# Autodesk Inventor assembly: multipurpose_distiller_assembly
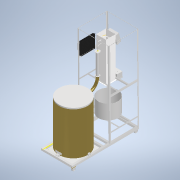
[picture p0: Inventor's stored thumbnail of the model, 180x180]
Saved by Autodesk Inventor 2020 (Build 240168000, 168)
## iProperties
Created: 2022-09-01
Part Number: multipurpose_distiller_assembly
Document SubType Name: Assembly
Designer: Intuito_PC
Author: Intuito_PC
## Documents named in this file (18)
- C:\Users\Intuito_PC\Desktop\academ\final_yr_project\auto_distiller\report_work\Project_Implementation_Report\CAD\multipurpose_distiller_assembly.iam
- C:\Users\Intuito_PC\Desktop\academ\final_yr_project\auto_distiller\report_work\Project_Implementation_Report\CAD\frame.ipt
- C:\Users\Intuito_PC\Desktop\academ\final_yr_project\auto_distiller\report_work\Project_Implementation_Report\CAD\still.ipt
- C:\Users\Intuito_PC\Desktop\academ\final_yr_project\auto_distiller\report_work\Project_Implementation_Report\CAD\fractionating_column.ipt
- C:\Users\Intuito_PC\Desktop\academ\final_yr_project\auto_distiller\report_work\Project_Implementation_Report\CAD\fractionating_column_cover.ipt
- C:\Users\Intuito_PC\Desktop\academ\final_yr_project\auto_distiller\report_work\Project_Implementation_Report\CAD\condenser.ipt
- C:\Users\Intuito_PC\Desktop\academ\final_yr_project\auto_distiller\report_work\Project_Implementation_Report\CAD\AC_heater_coil.ipt
- C:\Users\Intuito_PC\Desktop\academ\final_yr_project\auto_distiller\report_work\Project_Implementation_Report\CAD\AC_power_box.ipt
- C:\Users\Intuito_PC\Desktop\academ\final_yr_project\auto_distiller\report_work\Project_Implementation_Report\CAD\boiler_plates.ipt
- C:\Users\Intuito_PC\Desktop\academ\final_yr_project\auto_distiller\report_work\Project_Implementation_Report\CAD\control_panel_box.ipt
- C:\Users\Intuito_PC\Desktop\academ\final_yr_project\auto_distiller\report_work\Project_Implementation_Report\CAD\oil_water_separator.ipt
- C:\Users\Intuito_PC\Desktop\academ\final_yr_project\auto_distiller\report_work\Project_Implementation_Report\CAD\solar_power_buffer_battery.ipt
- C:\Users\Intuito_PC\Desktop\academ\final_yr_project\auto_distiller\report_work\Project_Implementation_Report\CAD\distilate_tank.ipt
- C:\Users\Intuito_PC\Desktop\academ\final_yr_project\auto_distiller\report_work\Project_Implementation_Report\CAD\still_cover.ipt
- C:\Users\Intuito_PC\Desktop\academ\final_yr_project\auto_distiller\report_work\Project_Implementation_Report\CAD\refractory_quarry_tile_pad.ipt
- C:\Users\Intuito_PC\Desktop\academ\final_yr_project\auto_distiller\report_work\Project_Implementation_Report\CAD\roller_coaster_wheel.ipt
- C:\Users\Intuito_PC\Desktop\academ\final_yr_project\auto_distiller\report_work\Project_Implementation_Report\CAD\radiator.ipt
- C:\Users\Intuito_PC\Desktop\academ\final_yr_project\auto_distiller\report_work\Project_Implementation_Report\CAD\radiator_fan.ipt
## Components (22 placed, 17 different names)
1. frame:1 — Mate:1, Mate:2, Mate:3, Mate:4, Mate:5, Mate:6, Mate:7, Mate:8, Mate:9, Mate:10, Mate:11, Mate:12, Mate:13, Mate:14, Mate:15, Mate:16, Mate:18, Mate:19, Mate:20
2. still:1 — Insert:1
3. fractionating_column:1
4. fractionating_column_cover:1
5. condenser:1
6. AC_heater_coil:1
7. AC_power_box:1
8. boiler_plates:1
9. control_panel_box:1 — Mate:1, Mate:2, Mate:3
10. oil_water_separator:1 — Mate:4, Mate:5, Mate:6
11. solar_power_buffer_battery:1 — Mate:7, Mate:8, Mate:9
12. distilate_tank:1 — Mate:10
13. still_cover:1 — Insert:1
14. refractory_quarry_tile_pad:1 — Mate:11, Mate:12, Mate:13, Mate:17
15. roller_coaster_wheel:1 — Mate:16
16. roller_coaster_wheel:2 — Mate:19
17. roller_coaster_wheel:3 — Mate:17
18. roller_coaster_wheel:4 — Mate:20
19. roller_coaster_wheel:5 — Mate:18
20. radiator:1 — Mate:14, Mate:15
21. radiator_fan:1
22. radiator_fan:2
## Relationships (21: Mate 20, Insert 1)
- Mate:1: frame:1 ↔ control_panel_box:1
- Mate:2: frame:1 ↔ control_panel_box:1
- Mate:3: frame:1 ↔ control_panel_box:1
- Mate:4: frame:1 ↔ oil_water_separator:1
- Mate:5: frame:1 ↔ oil_water_separator:1
- Mate:6: frame:1 ↔ oil_water_separator:1
- Mate:7: frame:1 ↔ solar_power_buffer_battery:1
- Mate:8: frame:1 ↔ solar_power_buffer_battery:1
- Mate:9: frame:1 ↔ solar_power_buffer_battery:1
- Mate:10: frame:1 ↔ distilate_tank:1
- Insert:1: still:1 ↔ still_cover:1
- Mate:11: frame:1 ↔ refractory_quarry_tile_pad:1
- Mate:12: frame:1 ↔ refractory_quarry_tile_pad:1
- Mate:13: frame:1 ↔ refractory_quarry_tile_pad:1
- Mate:14: frame:1 ↔ radiator:1
- Mate:15: frame:1 ↔ radiator:1
- Mate:16: frame:1 ↔ roller_coaster_wheel:1
- Mate:17: refractory_quarry_tile_pad:1 ↔ roller_coaster_wheel:3
- Mate:18: frame:1 ↔ roller_coaster_wheel:5
- Mate:19: frame:1 ↔ roller_coaster_wheel:2
- Mate:20: frame:1 ↔ roller_coaster_wheel:4
